# Autodesk Inventor assembly: Gear_test_2
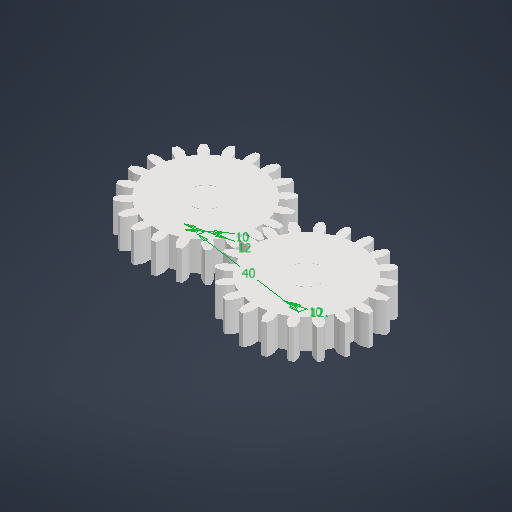
[picture p0: Inventor's stored thumbnail of the model, 512x512]
Saved by Autodesk Inventor 2026.2 (Build 302298000, 298)
## iProperties
Created: 2025-12-17
Part Number: Gear_test_2
Document SubType Name: Assembly
Designer: Cobble
Author: Cobble
## Documents named in this file (4)
- D:\CAD\Gear_test_2.iam
- D:\CAD\Test.ipt
- D:\CAD\40mm_20N_Gear.ipt
- D:\CAD\Gear_step1.ipt
## Components (5 placed, 3 different names)
1. 40mm_20N_Gear:1
2. 40mm_20N_Gear:2
3. Test:3 — Insert:9, Insert:10
4. Gear_step1:1 — Insert:9, Rotation:1
5. Gear_step1:2 — Insert:10, Rotation:1
## Relationships (3: Insert 2, RelateRotation 1)
- Insert:9: Test:3 ↔ Gear_step1:1
- Insert:10: Test:3 ↔ Gear_step1:2
- Rotation:1 [RelateRotation] (1 ul): Gear_step1:1 ↔ Gear_step1:2
